# Autodesk Inventor assembly: LiDAR_t
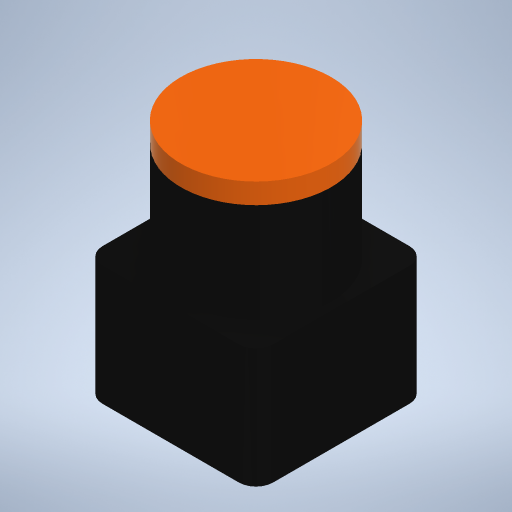
[picture p0: Inventor's stored thumbnail of the model, 512x512]
Saved by Autodesk Inventor 2023 (Build 270158000, 158)
## iProperties
Created: 2023-03-22
Part Number: LiDAR_t
Document SubType Name: Assembly
Designer: blueh
Author: blueh
## Documents named in this file (3)
- C:\Users\blueh\OneDrive - Kyushu University\2023NHK_RR_2ndvid\000_parts_zegi\sensor\LiDAR_t.iam
- C:\Users\blueh\Desktop\zip - コピー\ER_LIDER_1.ipt
- C:\Users\blueh\Desktop\zip - コピー\ER_LIDER_2.ipt
## Components (2 placed, 2 different names)
1. ER_LIDER_1:1
2. ER_LIDER_2:1
## Relationships (1: Insert 1)
- [Insert]: ER_LIDER_1:1 ↔ ER_LIDER_2:1
